# Autodesk Inventor assembly: Back_Wheel_Drive
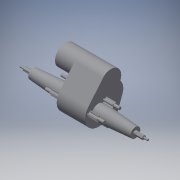
[picture p0: Inventor's stored thumbnail of the model, 180x180]
Saved by Autodesk Inventor 2019 (Build 230136000, 136)
## iProperties
Created: 2019-03-02
Part Number: Back_Wheel_Drive
Document SubType Name: Assembly
Designer: alarr
Author: alarr
## Documents named in this file (4)
- C:\Users\alarr\OneDrive\Documents\Inventor\Mr.Green\Back_Wheel_Drive.iam
- C:\Users\alarr\OneDrive\Documents\Inventor\Mr.Green\Back_Wheel_Drive.ipt
- C:\Users\alarr\OneDrive\Documents\Inventor\Mr.Green\Wheel_Pin.ipt
- C:\Users\alarr\OneDrive\Documents\Inventor\Mr.Green\Wheel_Pin_MIR.ipt
## Components (3 placed, 3 different names)
1. Back_Wheel_Drive:1 — Flush:1, Mate:1, Mate:2
2. Wheel_Pin:1 — Flush:1
3. Wheel_Pin_MIR:1 — Mate:1, Mate:2
## Relationships (3: Mate 2, Flush 1)
- Flush:1: Back_Wheel_Drive:1 ↔ Wheel_Pin:1
- Mate:1: Back_Wheel_Drive:1 ↔ Wheel_Pin_MIR:1
- Mate:2: Back_Wheel_Drive:1 ↔ Wheel_Pin_MIR:1
